# Autodesk Inventor assembly: A_AxialFluxMotor
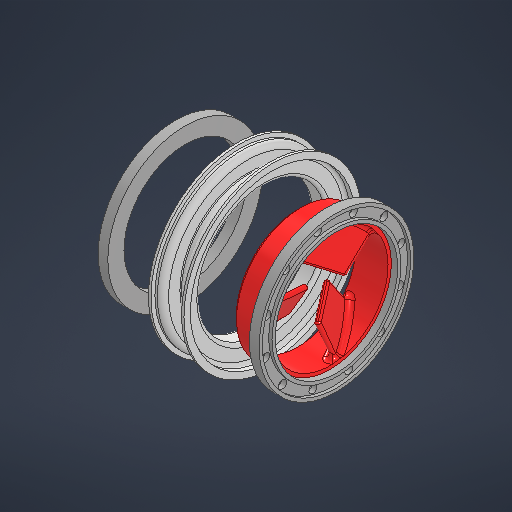
[picture p0: Inventor's stored thumbnail of the model, 512x512]
Saved by Autodesk Inventor 2026 (Build 300175000, 175)
## iProperties
Created: 2025-05-06
Part Number: A_AxialFluxMotor
Document SubType Name: Assembly
Designer: FAL
Author: FAL
## Documents named in this file (4)
- C:\Users\FAL\Desktop\git\AxialFluxMotor\A_AxialFluxMotor.iam
- C:\Users\FAL\Desktop\git\AxialFluxMotor\p_stratorCase.ipt
- C:\Users\FAL\Desktop\git\AxialFluxMotor\P_Rotor_A.ipt
- C:\Users\FAL\Desktop\git\AxialFluxMotor\P_magnetCase.ipt
## Components (4 placed, 3 different names)
1. p_stratorCase:1 — Passend:1, Passend:2, Fluchtend:1, Passend:3, Passend:4
2. P_Rotor_A:1 — Passend:3, Passend:5, Passend:6
3. P_magnetCase:1 — Passend:4, Passend:5
4. P_magnetCase:2 — Passend:6
## Relationships (7: Mate 6, Flush 1)
- Passend:1 [Mate]: p_stratorCase:1
- Passend:2 [Mate]: p_stratorCase:1
- Fluchtend:1 [Flush]: p_stratorCase:1
- Passend:3 [Mate]: p_stratorCase:1 ↔ P_Rotor_A:1
- Passend:4 [Mate]: p_stratorCase:1 ↔ P_magnetCase:1
- Passend:5 [Mate]: P_Rotor_A:1 ↔ P_magnetCase:1
- Passend:6 [Mate]: P_Rotor_A:1 ↔ P_magnetCase:2
